# Autodesk Inventor assembly: RCUv2-4Assy
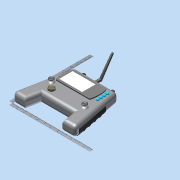
[picture p0: Inventor's stored thumbnail of the model, 180x180]
Saved by Autodesk Inventor 2011 SP1 (Build 150282100, 282)
## iProperties
Created: 2011-08-16
Part Number: RCUv2-4Assy
Document SubType Name: Assembly
Designer: dgitz
Author: dgitz
## Documents named in this file (4)
- C:\Dropbox\ICARUS\Remote Control Unit (RCU)\RCU v2\Design\RCUv2-4Assy.iam
- C:\Dropbox\ICARUS\Remote Control Unit (RCU)\RCU v2\Design\RCUv2-4\RCUAssy.iam
- C:\Dropbox\ICARUS\Remote Control Unit (RCU)\RCU v2\Design\Library\SpringSamsungGalaxySAssy.iam
- C:\Dropbox\ICARUS\Remote Control Unit (RCU)\RCU v2\Design\Imported Components\User Library-12 inch scale\Part24.ipt
## Components (4 placed, 3 different names)
1. RCUAssy:1 [sub-assembly] — Flush:2, Mate:1, Mate:2, Mate:5
2. SpringSamsungGalaxySAssy:1 [sub-assembly] — Mate:5
3. Part24:1 — Flush:1, Flush:2, Mate:1, Mate:2, Mate:3, Mate:4
4. Part24:2 — Flush:1, Mate:3, Mate:4
## Relationships (7: Mate 5, Flush 2)
- Flush:1: Part24:1 ↔ Part24:2
- Flush:2 (38.1 mm): RCUAssy:1 ↔ Part24:1
- Mate:1: RCUAssy:1 ↔ Part24:1
- Mate:2: RCUAssy:1 ↔ Part24:1
- Mate:3: Part24:1 ↔ Part24:2
- Mate:4: Part24:1 ↔ Part24:2
- Mate:5 (-12.7 mm): RCUAssy:1 ↔ SpringSamsungGalaxySAssy:1
